# Autodesk Inventor assembly: Leg_joint_roll
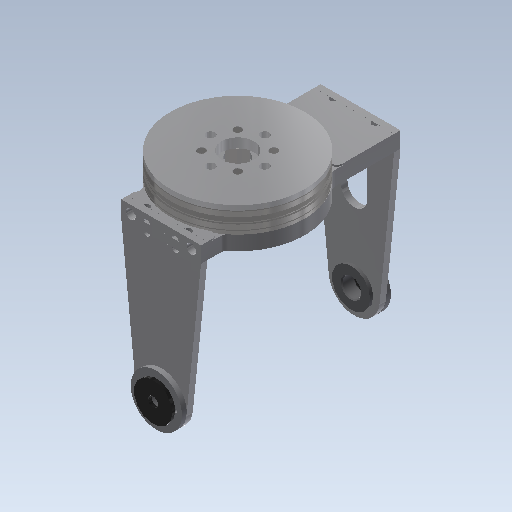
[picture p0: Inventor's stored thumbnail of the model, 512x512]
Saved by Autodesk Inventor 2020.4 (Build 244396000, 396)
## iProperties
Created: 2016-05-01
Part Number: Leg_joint_roll
Document SubType Name: Assembly
Designer: hiroaki
Mass: 101.489 g
Surface Area: 218.083 cm^2
Volume: 17.9148 cm^3
Density: 5.6651 g/cm^3
Author: hiroaki
## Documents named in this file (11)
- C:\Users\Masato\Documents\Inventor\CIT Brains_Inventor\OpenPlatform_ver3_0\LowerBody\Leg_joint_roll\Leg_Joint_roll.iam
- C:\Users\Masato\Documents\Inventor\CIT Brains_Inventor\OpenPlatform_ver3_0\LowerBody\Leg_joint_roll\Leg_Joint_roll_horizontal_01.ipt
- C:\Users\Masato\Documents\Inventor\CIT Brains_Inventor\OpenPlatform_ver3_0\Ready_Made\BA2542\BA2542.ipt
- C:\Users\Masato\Documents\Inventor\CIT Brains_Inventor\OpenPlatform_ver3_0\Thrust\Thrust_frame_01.ipt
- C:\Users\Masato\Documents\Inventor\CIT Brains_Inventor\OpenPlatform_ver3_0\Ready_Made\BA2542\BA2542_Washer.ipt
- C:\Users\Masato\Documents\Inventor\CIT Brains_Inventor\OpenPlatform_ver3_0\Ready_Made\MSU-306-03.ipt
- C:\Users\Masato\Documents\Inventor\CIT Brains_Inventor\OpenPlatform_ver3_0\LowerBody\Leg_joint_roll\Leg_Joint_roll_vertical_back.ipt
- C:\Users\Masato\Documents\Inventor\CIT Brains_Inventor\OpenPlatform_ver3_0\LowerBody\Leg_joint_roll\Leg_Joint_roll_vertical_front.ipt
- C:\Users\Masato\Documents\Inventor\CIT Brains_Inventor\OpenPlatform_ver3_0\Ready_Made\UUW-0312-10BH.ipt
- C:\Users\Masato\Documents\Inventor\CIT Brains_Inventor\OpenPlatform_ver3_0\Ready_Made\80F-0603.ipt
- C:\Users\Masato\Documents\Inventor\CIT Brains_Inventor\OpenPlatform_ver3_0\Ready_Made\LFW-0815.ipt
## Components (17 placed, 10 different names)
1. Leg_Joint_roll_horizontal_01:1 — 挿入:29, 挿入:31, 挿入:32, 挿入:33, 挿入:34, 挿入:38, 挿入:39, 挿入:40, 挿入:41
2. BA2542:1 — 挿入:30
3. BA2542:2 — 挿入:24
4. Thrust_frame_01:1 — 挿入:24, 挿入:35, 挿入:36, 挿入:37
5. BA2542_Washer:1 — 挿入:29, 挿入:30
6. MSU-306-03:1 — 挿入:31, 挿入:35
7. MSU-306-03:2 — 挿入:32, 挿入:36
8. MSU-306-03:3 — 挿入:33
9. MSU-306-03:4 — 挿入:34, 挿入:37
10. Leg_Joint_roll_vertical_back:1 — 挿入:40, 挿入:41, 挿入:42, 挿入:47
11. Leg_Joint_roll_vertical_front:1 — 挿入:38, 挿入:39, 挿入:43, 挿入:46
12. UUW-0312-10BH:3 — 挿入:45
13. UUW-0312-10BH:4 — 挿入:48
14. 80F-0603:1 — 挿入:43
15. 80F-0603:2 — 挿入:42
16. LFW-0815:1 — 挿入:45, 挿入:46
17. LFW-0815:2 — 挿入:47, 挿入:48
## Relationships (20: Insert 20)
- 挿入:24 [Insert]: BA2542:2 ↔ Thrust_frame_01:1
- 挿入:29 [Insert]: Leg_Joint_roll_horizontal_01:1 ↔ BA2542_Washer:1
- 挿入:30 [Insert]: BA2542:1 ↔ BA2542_Washer:1
- 挿入:31 [Insert]: Leg_Joint_roll_horizontal_01:1 ↔ MSU-306-03:1
- 挿入:32 [Insert]: Leg_Joint_roll_horizontal_01:1 ↔ MSU-306-03:2
- 挿入:33 [Insert]: Leg_Joint_roll_horizontal_01:1 ↔ MSU-306-03:3
- 挿入:34 [Insert]: Leg_Joint_roll_horizontal_01:1 ↔ MSU-306-03:4
- 挿入:35 [Insert]: Thrust_frame_01:1 ↔ MSU-306-03:1
- 挿入:36 [Insert]: Thrust_frame_01:1 ↔ MSU-306-03:2
- 挿入:37 [Insert]: Thrust_frame_01:1 ↔ MSU-306-03:4
- 挿入:38 [Insert]: Leg_Joint_roll_horizontal_01:1 ↔ Leg_Joint_roll_vertical_front:1
- 挿入:39 [Insert]: Leg_Joint_roll_horizontal_01:1 ↔ Leg_Joint_roll_vertical_front:1
- 挿入:40 [Insert]: Leg_Joint_roll_horizontal_01:1 ↔ Leg_Joint_roll_vertical_back:1
- 挿入:41 [Insert]: Leg_Joint_roll_horizontal_01:1 ↔ Leg_Joint_roll_vertical_back:1
- 挿入:42 [Insert]: Leg_Joint_roll_vertical_back:1 ↔ 80F-0603:2
- 挿入:43 [Insert]: Leg_Joint_roll_vertical_front:1 ↔ 80F-0603:1
- 挿入:45 [Insert]: UUW-0312-10BH:3 ↔ LFW-0815:1
- 挿入:46 [Insert]: Leg_Joint_roll_vertical_front:1 ↔ LFW-0815:1
- 挿入:47 [Insert]: Leg_Joint_roll_vertical_back:1 ↔ LFW-0815:2
- 挿入:48 [Insert]: UUW-0312-10BH:4 ↔ LFW-0815:2
